# Autodesk Inventor assembly: 4x18BoltWasher
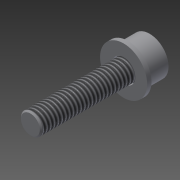
[picture p0: Inventor's stored thumbnail of the model, 180x180]
Saved by Autodesk Inventor 2015 (Build 190159000, 159)
## iProperties
Created: 2014-02-08
Part Number: 4x18BoltWasher
Document SubType Name: Assembly
Designer: Jack
Author: Jack
## Documents named in this file (3)
- C:\Users\Jack\Sync\MendelMax1.5\InventorParts\Hardware\BoltWashers\4x18BoltWasher.iam
- C:\Users\Jack\Sync\MendelMax1.5\InventorParts\Hardware\Bolts\M4x18SHCS.ipt
- C:\Users\Jack\Sync\MendelMax1.5\InventorParts\Hardware\Washers\M4Washer.ipt
## Components (2 placed, 2 different names)
1. M4x18SHCS:1 — Mate:1, Mate:2
2. M4Washer:1 — Mate:1, Mate:2
## Relationships (2: Mate 2)
- Mate:1: M4x18SHCS:1 ↔ M4Washer:1
- Mate:2: M4x18SHCS:1 ↔ M4Washer:1
